# Autodesk Inventor assembly: Chassis
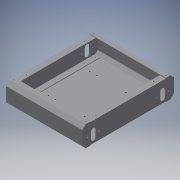
[picture p0: Inventor's stored thumbnail of the model, 180x180]
Saved by Autodesk Inventor 2016 (Build 200138000, 138)
## iProperties
Created: 2015-08-06
Part Number: Chassis
Document SubType Name: Assembly
Designer: lachesis
Author: lachesis
## Documents named in this file (4)
- C:\Users\lachesis\git\Swarmie-Build\Swarmie Assembly\Assemblies\Chassis.iam
- C:\Users\lachesis\git\Swarmie-Build\Swarmie Assembly\Parts\ChassisMainBracket.ipt
- C:\Users\lachesis\git\Swarmie-Build\Swarmie Assembly\Parts\ChassisSideBracket.ipt
- C:\Users\lachesis\git\Swarmie-Build\Swarmie Assembly\Parts\BottomPlate.ipt
## Components (5 placed, 3 different names)
1. ChassisMainBracket:1 — Rigid:1, Rigid:4
2. ChassisMainBracket:2 — Rigid:2, Rigid:3
3. ChassisSideBracket:1 — Rigid:1, Rigid:2, Rotational:1
4. ChassisSideBracket:2 — Rigid:3, Rigid:4
5. BottomPlate:1 — Rotational:1
## Relationships (5: WeldJoint 4, RevoluteJoint 1)
- Rigid:1 [WeldJoint]: ChassisMainBracket:1 ↔ ChassisSideBracket:1
- Rigid:2 [WeldJoint]: ChassisMainBracket:2 ↔ ChassisSideBracket:1
- Rigid:3 [WeldJoint]: ChassisMainBracket:2 ↔ ChassisSideBracket:2
- Rigid:4 [WeldJoint]: ChassisMainBracket:1 ↔ ChassisSideBracket:2
- Rotational:1 [RevoluteJoint]: ChassisSideBracket:1 ↔ BottomPlate:1
